# Autodesk Inventor assembly: Sandbox
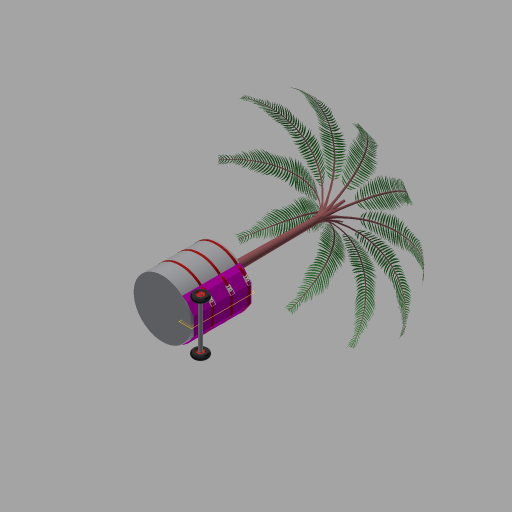
[picture p0: Inventor's stored thumbnail of the model, 512x512]
Saved by Autodesk Inventor 2023.2 (Build 272271000, 271)
## iProperties
Created: 2023-02-01
Part Number: Sandbox
Material: Generisch
Document SubType Name: Assembly
Designer: Raoul Messerli
Author: Raoul Messerli
## Documents named in this file (7)
- E:\GitHub\Pflanzenwagen\20_Inventor\40_Baugruppen\Sandbox.iam
- E:\GitHub\Pflanzenwagen\20_Inventor\10_Vorlage\Palme.iam
- E:\GitHub\Pflanzenwagen\20_Inventor\20_Einkaufteile\RatchetStrap\RatchetStrap\RatchetStrap.iam
- E:\GitHub\Pflanzenwagen\20_Inventor\30_Fertigungsteile\Blech1.ipt
- E:\GitHub\Pflanzenwagen\20_Inventor\20_Einkaufteile\RatchetStrap\Strap for Pflanzenwagen.ipt
- E:\GitHub\Pflanzenwagen\20_Inventor\20_Einkaufteile\Wheel.ipt
- E:\GitHub\Pflanzenwagen\20_Inventor\30_Fertigungsteile\Achse.ipt
## Components (11 placed, 6 different names)
1. Strap for Pflanzenwagen:1 — Passend:7, Fluchtend:9, Passend:8
2. Strap for Pflanzenwagen:2 — Passend:9, Fluchtend:10, Passend:10
3. Strap for Pflanzenwagen:3 — Passend:11, Fluchtend:11, Passend:12
4. Palme:1 [sub-assembly] — Fluchtend:1, Fluchtend:2, Tangential:1, Fluchtend:3, Fluchtend:4, Fluchtend:5, Passend:13, Passend:14
5. Blech1:1 — Fluchtend:1, Fluchtend:2, Tangential:1, Fluchtend:6, Passend:1, Passend:2, Passend:3, Fluchtend:7, Passend:4, Passend:5, Fluchtend:8, Passend:6, Passend:10, Tangential:2
6. RatchetStrap:1 [sub-assembly] — Fluchtend:6, Passend:1, Passend:2, Passend:8
7. RatchetStrap:2 [sub-assembly] — Passend:3, Fluchtend:7, Passend:4
8. RatchetStrap:3 [sub-assembly] — Passend:5, Fluchtend:8, Passend:6, Passend:12
9. Achse:1 — Passend:13, Passend:14, Tangential:2, Passend:15, Passend:16, Passend:17, Passend:18
10. Wheel:2 — Passend:17, Passend:18
11. Wheel:3 — Passend:15, Passend:16
## Relationships (31: Mate 18, Flush 11, Tangent 2)
- Fluchtend:1 [Flush]: Palme:1 ↔ Blech1:1
- Fluchtend:2 [Flush]: Palme:1 ↔ Blech1:1
- Tangential:1: Palme:1 ↔ Blech1:1
- Fluchtend:3 [Flush]: Palme:1
- Fluchtend:4 [Flush]: Palme:1
- Fluchtend:5 [Flush]: Palme:1
- Fluchtend:6 [Flush]: Blech1:1 ↔ RatchetStrap:1
- Passend:1 [Mate]: Blech1:1 ↔ RatchetStrap:1
- Passend:2 [Mate]: Blech1:1 ↔ RatchetStrap:1
- Passend:3 [Mate]: Blech1:1 ↔ RatchetStrap:2
- Fluchtend:7 [Flush]: Blech1:1 ↔ RatchetStrap:2
- Passend:4 [Mate]: Blech1:1 ↔ RatchetStrap:2
- Passend:5 [Mate]: Blech1:1 ↔ RatchetStrap:3
- Fluchtend:8 [Flush]: Blech1:1 ↔ RatchetStrap:3
- Passend:6 [Mate]: Blech1:1 ↔ RatchetStrap:3
- Passend:7 [Mate]: Strap for Pflanzenwagen:1
- Fluchtend:9 [Flush]: Strap for Pflanzenwagen:1
- Passend:8 [Mate]: Strap for Pflanzenwagen:1 ↔ RatchetStrap:1
- Passend:9 [Mate]: Strap for Pflanzenwagen:2
- Fluchtend:10 [Flush]: Strap for Pflanzenwagen:2
- Passend:10 [Mate]: Strap for Pflanzenwagen:2 ↔ Blech1:1
- Passend:11 [Mate]: Strap for Pflanzenwagen:3
- Fluchtend:11 [Flush]: Strap for Pflanzenwagen:3
- Passend:12 [Mate]: Strap for Pflanzenwagen:3 ↔ RatchetStrap:3
- Passend:13 [Mate] (-420 mm): Palme:1 ↔ Achse:1
- Passend:14 [Mate] (400 mm): Palme:1 ↔ Achse:1
- Tangential:2: Blech1:1 ↔ Achse:1
- Passend:15 [Mate]: Achse:1 ↔ Wheel:3
- Passend:16 [Mate]: Achse:1 ↔ Wheel:3
- Passend:17 [Mate]: Achse:1 ↔ Wheel:2
- Passend:18 [Mate]: Achse:1 ↔ Wheel:2
